# Autodesk Inventor assembly: TNS_Greiferbacke_MA_Jun
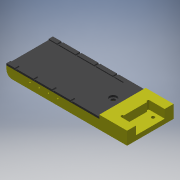
[picture p0: Inventor's stored thumbnail of the model, 180x180]
Saved by Autodesk Inventor 2017 (Build 210142000, 142)
## iProperties
Created: 2018-03-14
Part Number: TNS_Greiferbacke_MA_Jun
Document SubType Name: Assembly
Designer: uoehq
Author: uoehq
## Documents named in this file (3)
- C:\Users\uoehq\Documents\Git\Feature_Embedding\Greifer\3d_datei\TNS_Greiferbacke_MA_Jun.iam
- C:\Users\uoehq\Documents\Git\Feature_Embedding\Greifer\3d_datei\TNS_Greiferbacke_MA_Jun_T1.ipt
- C:\Users\uoehq\Documents\Git\Feature_Embedding\Greifer\3d_datei\TNS_Greiferbacke_MA_Jun_T2.ipt
## Components (2 placed, 2 different names)
1. TNS_Greiferbacke_MA_Jun_T1:1 — Mate:1, Mate:2, Flush:1
2. TNS_Greiferbacke_MA_Jun_T2:1 — Mate:1, Mate:2, Flush:1
## Relationships (3: Mate 2, Flush 1)
- Mate:1: TNS_Greiferbacke_MA_Jun_T1:1 ↔ TNS_Greiferbacke_MA_Jun_T2:1
- Mate:2: TNS_Greiferbacke_MA_Jun_T1:1 ↔ TNS_Greiferbacke_MA_Jun_T2:1
- Flush:1: TNS_Greiferbacke_MA_Jun_T1:1 ↔ TNS_Greiferbacke_MA_Jun_T2:1
